# Autodesk Inventor assembly: Cableholder+Magnets
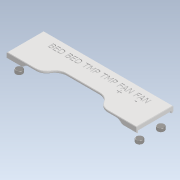
[picture p0: Inventor's stored thumbnail of the model, 180x180]
Saved by Autodesk Inventor 2022.1 (Build 261234020, 234B)
## iProperties
Created: 2022-07-24
Part Number: Cableholder+Magnets
Document SubType Name: Assembly
Designer: Rama
Author: Rama
## Documents named in this file (3)
- C:\Users\Rama\Desktop\GitHub\Voron-2-Mods\Mandalaroseworks\BedPan\CAD\SRC\Manual_Helpers\Cableholder+Magnets.iam
- C:\Users\Rama\Desktop\GitHub\Voron-2-Mods\Mandalaroseworks\BedPan\CAD\SRC\Cableholder\Cableholder.ipt
- C:\Users\Rama\Desktop\Work Priv\Klicky\6x3 Magnet.ipt
## Components (5 placed, 2 different names)
1. Cableholder:1 — Passend:1, Passend:2, Passend:3, Passend:4
2. 6x3 Magnet:1 — Passend:3
3. 6x3 Magnet:2 — Passend:2
4. 6x3 Magnet:3 — Passend:1
5. 6x3 Magnet:4 — Passend:4
## Relationships (7: Mate 4, Flush 3)
- [Flush]: 6x3 Magnet:2 ↔ 6x3 Magnet:3
- [Flush]: 6x3 Magnet:1 ↔ 6x3 Magnet:4
- [Flush]: 6x3 Magnet:3 ↔ 6x3 Magnet:4
- Passend:1 [Mate]: Cableholder:1 ↔ 6x3 Magnet:3
- Passend:2 [Mate]: Cableholder:1 ↔ 6x3 Magnet:2
- Passend:3 [Mate]: Cableholder:1 ↔ 6x3 Magnet:1
- Passend:4 [Mate]: Cableholder:1 ↔ 6x3 Magnet:4
